# Autodesk Inventor assembly: Trolley
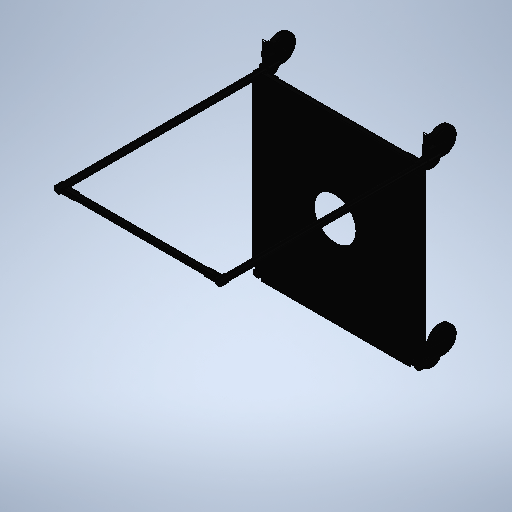
[picture p0: Inventor's stored thumbnail of the model, 512x512]
Saved by Autodesk Inventor 2025.2 (Build 292293000, 293)
## iProperties
Created: 2025-05-24
Part Number: Trolley
Description: STEP AP214
Document SubType Name: Assembly
Designer: Musa Gamal
Sending System: SolidWorks 2023
Preprocessor: SwSTEP 2.0
Title: Trolley.STEP
Revision Number: ANY
## Documents named in this file (2)
- D:\ASU\senior 1\semster 2\Advanced Manufacturing Technology & Prototyping\Project\Trolley\Trolley\Trolley.iam
- D:\ASU\senior 1\semster 2\Advanced Manufacturing Technology & Prototyping\Project\Trolley\Trolley\TROLI.step.iam
## Components (1 placed, 1 different names)
1. TROLI.step_1 [sub-assembly] — Angle:1, Tangent:1
## Relationships (2: Angle 1, Tangent 1)
- Angle:1 (0 deg): TROLI.step_1
- Tangent:1: TROLI.step_1
